# Autodesk Inventor assembly: IMUTracker
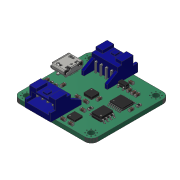
[picture p0: Inventor's stored thumbnail of the model, 180x180]
Saved by Autodesk Inventor 2019.4 (Build 234330000, 330)
## iProperties
Created: 2019-02-04
Part Number: IMUTracker
Material: 一般
Description: FreeCAD Model
Document SubType Name: Assembly
Designer: y6tada
Authority: Unknown
Sending System: FreeCAD
Preprocessor: Open CASCADE STEP processor 7.2
Title: /Users/user/Library/Mobile Documents/com~apple~CloudDocs/filepost/IMUCapture/IMUCapture.step
Author: Author
## Documents named in this file (2)
- C:\Workspace\QUIKS\Hardware\IMUTracker\Circuit\IMUTracker_Inveotor_model\IMUTracker.iam
- C:\Workspace\QUIKS\Hardware\IMUTracker\Circuit\IMUTracker_Inveotor_model\Step_Models.iam
## Components (1 placed, 1 different names)
1. 60 [sub-assembly] — フラッシュ:1, フラッシュ:2, メイト:1
## Relationships (3: Flush 2, Mate 1)
- フラッシュ:1 [Flush] (15 mm): 60
- フラッシュ:2 [Flush] (15 mm): 60
- メイト:1 [Mate]: 60
